# Autodesk Inventor assembly: Universal Joint
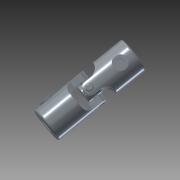
[picture p0: Inventor's stored thumbnail of the model, 180x180]
Saved by Autodesk Inventor 2016 SP2 (Build 200236200, 236)
## iProperties
Created: 2012-02-01
Part Number: Universal Joint
Description: STEP AP203
Document SubType Name: Assembly
Designer: Jacob
Sending System: SolidWorks 2011
Preprocessor: SwSTEP 2.0
Title: 276-2045-002-000 Rev2.STEP
Revision Number: ANY
## Documents named in this file (5)
- D:\Users\Owner\Desktop\VEX Parts\Imperial\Motion\Universal Joint.iam
- D:\Users\Owner\Desktop\Inventor Files\VEX Parts\Imperial\Motion\Components\276-2045-002-003 Rev1.ipt
- D:\Users\Owner\Desktop\Inventor Files\VEX Parts\Imperial\Motion\Components\276-2045-002-004 Rev1.ipt
- D:\Users\Owner\Desktop\Inventor Files\VEX Parts\Imperial\Motion\Components\276-2045-002-002 Rev2.ipt
- D:\Users\Owner\Desktop\Inventor Files\VEX Parts\Imperial\Motion\Components\276-2045-002-001 Rev1.ipt
## Components (7 placed, 7 different names)
1. 276-2045-002-003 Rev1_1 — Mate:2, Insert:1, Mate:6
2. 276-2045-002-004 Rev1_2 — Mate:9, Insert:3
3. 276-2045-002-002 Rev2_3 — Mate:5, Mate:6, Mate:7, Mate:8
4. 276-2045-002-004 Rev1_4 — Mate:3, Mate:4
5. 276-2045-002-001 Rev1_5 — Mate:1, Insert:2, Mate:7, Mate:9, Insert:3
6. 276-2045-002-003 Rev1_6 — Mate:1, Insert:2, Mate:5
7. 276-2045-002-001 Rev1_7 — Mate:2, Mate:3, Mate:4, Insert:1, Mate:8
## Relationships (12: Mate 9, Insert 3)
- Mate:1: 276-2045-002-001 Rev1_5 ↔ 276-2045-002-003 Rev1_6
- Mate:2: 276-2045-002-003 Rev1_1 ↔ 276-2045-002-001 Rev1_7
- Mate:3: 276-2045-002-004 Rev1_4 ↔ 276-2045-002-001 Rev1_7
- Mate:4 (-5.08 mm): 276-2045-002-004 Rev1_4 ↔ 276-2045-002-001 Rev1_7
- Insert:1 (-2.159 mm): 276-2045-002-003 Rev1_1 ↔ 276-2045-002-001 Rev1_7
- Insert:2 (-2.159 mm): 276-2045-002-001 Rev1_5 ↔ 276-2045-002-003 Rev1_6
- Mate:5: 276-2045-002-002 Rev2_3 ↔ 276-2045-002-003 Rev1_6
- Mate:6: 276-2045-002-003 Rev1_1 ↔ 276-2045-002-002 Rev2_3
- Mate:7 (2.54 mm): 276-2045-002-002 Rev2_3 ↔ 276-2045-002-001 Rev1_5
- Mate:8 (2.54 mm): 276-2045-002-002 Rev2_3 ↔ 276-2045-002-001 Rev1_7
- Mate:9: 276-2045-002-004 Rev1_2 ↔ 276-2045-002-001 Rev1_5
- Insert:3 (-3.302 mm): 276-2045-002-004 Rev1_2 ↔ 276-2045-002-001 Rev1_5
